# Autodesk Inventor assembly: ASY ДМФ 0100 Барабан
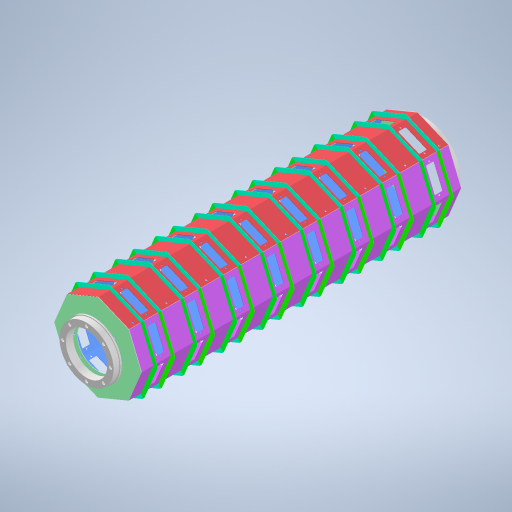
[picture p0: Inventor's stored thumbnail of the model, 512x512]
Saved by Autodesk Inventor 2024.2 (Build 282272000, 272)
## iProperties
Created: 2024-04-28
Part Number: ASY ДМФ 0100 Барабан
Document SubType Name: Assembly
Designer: pokla
Author: pokla
## Documents named in this file (25)
- C:\Users\admin\Documents\Inventor\DMF-Disk-Micro-Filter\ASY ДМФ 0100 Барабан.iam
- C:\Users\admin\Documents\Inventor\DMF-Disk-Micro-Filter\ДМФ 01 21 Барабан торец НОС.ipt
- C:\Users\admin\Documents\Inventor\DMF-Disk-Micro-Filter\ДМФ 01 13 Барабан Лист лев брт.ipt
- C:\Users\admin\Documents\Inventor\DMF-Disk-Micro-Filter\ДМФ 01 14 Барабан Лист прав брт.ipt
- C:\Users\admin\Documents\Inventor\DMF-Disk-Micro-Filter\ДМФ 01 31 Барабан Опорное кольцо НОС.ipt
- C:\Users\admin\Documents\Inventor\DMF-Disk-Micro-Filter\ДМФ 01 17 опора крышки.ipt
- C:\Users\admin\Documents\Inventor\DMF-Disk-Micro-Filter\ДМС 000 размеры.ipt
- C:\Users\admin\Documents\Inventor\DMF-Disk-Micro-Filter\ДМФ 01 41 Шестерня ведомая.ipt
- C:\Users\admin\Documents\Inventor\DMF-Disk-Micro-Filter\ДМФ 01 12 Барабан усилитель.ipt
- C:\Users\admin\Documents\Inventor\DMF-Disk-Micro-Filter\ASY ДМФ 010 крышка.iam
- C:\Users\admin\Documents\Inventor\DMF-Disk-Micro-Filter\ДМФ 01 32 Барабан Опорное кольцо КОРМА.ipt
- C:\Users\admin\Documents\Inventor\DMF-Disk-Micro-Filter\ДМФ 01 22 Барабан торец КОРМА.ipt
- C:\Users\admin\Documents\Inventor\DMF-Disk-Micro-Filter\ASY ДМФ 01 50 Кассета.iam
- ДМС 103 Опорное кольцо вала хвост.ipt
- C:\Users\admin\Documents\Inventor\DMF-Disk-Micro-Filter\ДМС 101 Барабан торец.ipt
- C:\Users\admin\Documents\Inventor\DMF-Disk-Micro-Filter\ДМФ 011 Барабан Лист левый борт.ipt
- C:\Users\admin\Documents\Inventor\DMF-Disk-Micro-Filter\ДМФ 012 Барабан Лист прав брт.ipt
- C:\Users\admin\Documents\Inventor\DMF-Disk-Micro-Filter\ДМС 102 Опорное кольцо вала перед.ipt
- C:\Users\admin\Documents\Inventor\DMF-Disk-Micro-Filter\ДМС 103 Полка для крышки.ipt
- C:\Users\admin\Documents\Inventor\DMF-Disk-Micro-Filter\ДМС 105 Шестерня ведомая.ipt
- C:\Users\admin\Documents\Inventor\DMF-Disk-Micro-Filter\ДМФ 0112 Сектор кольца усилителя барабана_CPY.ipt
- C:\Users\admin\Documents\Inventor\DMF-Disk-Micro-Filter\ASY ДМФ 0110 крышка галка.iam
- C:\Users\admin\Documents\Inventor\DMF-Disk-Micro-Filter\ДМС 103 Опорное кольцо вала хвост.ipt.ipt
- C:\Users\admin\Documents\Inventor\DMF-Disk-Micro-Filter\ДМС 101 Барабан торец зад.ipt
- C:\Users\admin\Documents\Inventor\DMF-Disk-Micro-Filter\ASY ДМФ 0120 Кассета.iam
## Components (123 placed, 12 different names)
1. ДМС 000 размеры:1
2. ДМС 102 Опорное кольцо вала перед:1 — Mate:1, Mate:2, Rotational:4, Mate:6, Rotational:5
3. ДМС 103 Опорное кольцо вала хвост.ipt:1 — Rotational:7, Mate:14
4. ДМС 101 Барабан торец:2 — Rotational:5, Mate:7, Rigid:15, Rigid:16, Mate:8, Flush:1, Flush:2, Mate:9, Flush:3, Flush:4, Mate:10, Flush:5, Flush:6, Rotational:6
5. ДМФ 011 Барабан Лист левый борт:1 — Rigid:15, Mate:12, Flush:7
6. ДМФ 012 Барабан Лист прав брт:1 — Rigid:16, Mate:11
7. ДМС 103 Полка для крышки:1 — Mate:9, Flush:3, Flush:4
8. ДМС 103 Полка для крышки:2 — Mate:8, Flush:1, Flush:2
9. ДМС 105 Шестерня ведомая:1 — Rotational:4, Mate:6
10. ASY ДМФ 0110 крышка галка:1 [sub-assembly] — Mate:10, Flush:5, Flush:6
11. ДМС 101 Барабан торец зад:1 — Rotational:6, Mate:13, Rotational:7
12. ДМФ 0112 Сектор кольца усилителя барабана_CPY:4 — Rigid:10
13. ДМФ 0112 Сектор кольца усилителя барабана_CPY:1 — Rigid:8
14. ДМФ 0112 Сектор кольца усилителя барабана_CPY:5 — Rigid:10, Rigid:11, Rigid:14
15. ДМФ 0112 Сектор кольца усилителя барабана_CPY:2 — Rigid:8, Rigid:9, Rigid:14
16. ДМФ 0112 Сектор кольца усилителя барабана_CPY:3 — Rigid:9, Mate:12
17. ДМФ 0112 Сектор кольца усилителя барабана_CPY:6 — Rigid:11
18. ДМФ 0112 Сектор кольца усилителя барабана_CPY:7
19. ДМФ 0112 Сектор кольца усилителя барабана_CPY:8
20. ДМФ 0112 Сектор кольца усилителя барабана_CPY:21
21. ДМФ 0112 Сектор кольца усилителя барабана_CPY:28
22. ДМФ 0112 Сектор кольца усилителя барабана_CPY:35
23. ДМФ 0112 Сектор кольца усилителя барабана_CPY:42
24. ДМФ 0112 Сектор кольца усилителя барабана_CPY:9
25. ДМФ 0112 Сектор кольца усилителя барабана_CPY:10
26. ДМФ 0112 Сектор кольца усилителя барабана_CPY:22
27. ДМФ 0112 Сектор кольца усилителя барабана_CPY:29
28. ДМФ 0112 Сектор кольца усилителя барабана_CPY:36
29. ДМФ 0112 Сектор кольца усилителя барабана_CPY:43
30. ДМФ 0112 Сектор кольца усилителя барабана_CPY:11
31. ДМФ 0112 Сектор кольца усилителя барабана_CPY:12
32. ДМФ 0112 Сектор кольца усилителя барабана_CPY:23
33. ДМФ 0112 Сектор кольца усилителя барабана_CPY:30
34. ДМФ 0112 Сектор кольца усилителя барабана_CPY:37
35. ДМФ 0112 Сектор кольца усилителя барабана_CPY:44
36. ДМФ 0112 Сектор кольца усилителя барабана_CPY:13
37. ДМФ 0112 Сектор кольца усилителя барабана_CPY:14
38. ДМФ 0112 Сектор кольца усилителя барабана_CPY:24
39. ДМФ 0112 Сектор кольца усилителя барабана_CPY:31
40. ДМФ 0112 Сектор кольца усилителя барабана_CPY:38
41. ДМФ 0112 Сектор кольца усилителя барабана_CPY:45
42. ДМФ 0112 Сектор кольца усилителя барабана_CPY:15
43. ДМФ 0112 Сектор кольца усилителя барабана_CPY:16
44. ДМФ 0112 Сектор кольца усилителя барабана_CPY:25
45. ДМФ 0112 Сектор кольца усилителя барабана_CPY:32
46. ДМФ 0112 Сектор кольца усилителя барабана_CPY:39
47. ДМФ 0112 Сектор кольца усилителя барабана_CPY:46
48. ДМФ 0112 Сектор кольца усилителя барабана_CPY:17
49. ДМФ 0112 Сектор кольца усилителя барабана_CPY:18
50. ДМФ 0112 Сектор кольца усилителя барабана_CPY:26
51. ДМФ 0112 Сектор кольца усилителя барабана_CPY:33
52. ДМФ 0112 Сектор кольца усилителя барабана_CPY:40
53. ДМФ 0112 Сектор кольца усилителя барабана_CPY:47
54. ДМФ 0112 Сектор кольца усилителя барабана_CPY:19 — Mate:11
55. ДМФ 0112 Сектор кольца усилителя барабана_CPY:20
56. ДМФ 0112 Сектор кольца усилителя барабана_CPY:27
57. ДМФ 0112 Сектор кольца усилителя барабана_CPY:34
58. ДМФ 0112 Сектор кольца усилителя барабана_CPY:41
59. ДМФ 0112 Сектор кольца усилителя барабана_CPY:48 — Flush:7
60. ASY ДМФ 0120 Кассета:1 [sub-assembly]
61. ASY ДМФ 0120 Кассета:2 [sub-assembly]
62. ASY ДМФ 0120 Кассета:3 [sub-assembly]
63. ASY ДМФ 0120 Кассета:4 [sub-assembly]
64. ASY ДМФ 0120 Кассета:5 [sub-assembly]
65. ASY ДМФ 0120 Кассета:6 [sub-assembly]
66. ASY ДМФ 0120 Кассета:7 [sub-assembly]
67. ASY ДМФ 0120 Кассета:8 [sub-assembly]
68. ASY ДМФ 0120 Кассета:9 [sub-assembly]
69. ASY ДМФ 0120 Кассета:10 [sub-assembly]
70. ASY ДМФ 0120 Кассета:11 [sub-assembly]
71. ASY ДМФ 0120 Кассета:12 [sub-assembly]
72. ASY ДМФ 0120 Кассета:13 [sub-assembly]
73. ASY ДМФ 0120 Кассета:14 [sub-assembly]
74. ASY ДМФ 0120 Кассета:15 [sub-assembly]
75. ASY ДМФ 0120 Кассета:16 [sub-assembly]
76. ASY ДМФ 0120 Кассета:17 [sub-assembly]
77. ASY ДМФ 0120 Кассета:18 [sub-assembly]
78. ASY ДМФ 0120 Кассета:19 [sub-assembly]
79. ASY ДМФ 0120 Кассета:20 [sub-assembly]
80. ASY ДМФ 0120 Кассета:21 [sub-assembly]
81. ASY ДМФ 0120 Кассета:22 [sub-assembly]
82. ASY ДМФ 0120 Кассета:23 [sub-assembly]
83. ASY ДМФ 0120 Кассета:24 [sub-assembly]
84. ASY ДМФ 0120 Кассета:25 [sub-assembly]
85. ASY ДМФ 0120 Кассета:26 [sub-assembly]
86. ASY ДМФ 0120 Кассета:27 [sub-assembly]
87. ASY ДМФ 0120 Кассета:28 [sub-assembly]
88. ASY ДМФ 0120 Кассета:29 [sub-assembly]
89. ASY ДМФ 0120 Кассета:30 [sub-assembly]
90. ASY ДМФ 0120 Кассета:31 [sub-assembly]
91. ASY ДМФ 0120 Кассета:32 [sub-assembly]
92. ASY ДМФ 0120 Кассета:33 [sub-assembly]
93. ASY ДМФ 0120 Кассета:34 [sub-assembly]
94. ASY ДМФ 0120 Кассета:35 [sub-assembly]
95. ASY ДМФ 0120 Кассета:36 [sub-assembly]
96. ASY ДМФ 0120 Кассета:37 [sub-assembly]
97. ASY ДМФ 0120 Кассета:38 [sub-assembly]
98. ASY ДМФ 0120 Кассета:39 [sub-assembly]
99. ASY ДМФ 0120 Кассета:40 [sub-assembly]
100. ASY ДМФ 0120 Кассета:41 [sub-assembly]
101. ASY ДМФ 0120 Кассета:42 [sub-assembly]
102. ASY ДМФ 0120 Кассета:43 [sub-assembly]
103. ASY ДМФ 0120 Кассета:44 [sub-assembly]
104. ASY ДМФ 0120 Кассета:45 [sub-assembly]
105. ASY ДМФ 0120 Кассета:46 [sub-assembly]
106. ASY ДМФ 0120 Кассета:47 [sub-assembly]
107. ASY ДМФ 0120 Кассета:48 [sub-assembly]
108. ASY ДМФ 0120 Кассета:49 [sub-assembly]
109. ASY ДМФ 0120 Кассета:50 [sub-assembly]
110. ASY ДМФ 0120 Кассета:51 [sub-assembly]
111. ASY ДМФ 0120 Кассета:52 [sub-assembly]
112. ASY ДМФ 0120 Кассета:53 [sub-assembly]
113. ASY ДМФ 0120 Кассета:54 [sub-assembly]
114. ASY ДМФ 0120 Кассета:55 [sub-assembly]
115. ASY ДМФ 0120 Кассета:56 [sub-assembly]
116. ASY ДМФ 0120 Кассета:57 [sub-assembly]
117. ASY ДМФ 0120 Кассета:58 [sub-assembly]
118. ASY ДМФ 0120 Кассета:59 [sub-assembly]
119. ASY ДМФ 0120 Кассета:60 [sub-assembly]
120. ASY ДМФ 0120 Кассета:61 [sub-assembly]
121. ASY ДМФ 0120 Кассета:62 [sub-assembly]
122. ASY ДМФ 0120 Кассета:63 [sub-assembly]
123. ASY ДМФ 0120 Кассета:64 [sub-assembly]
## Component patterns: (8 elements, first: ДМФ 0112 Сектор кольца усилителя барабана_CPY:4 + ДМФ 0112 Сектор кольца усилителя барабана_CPY:1 + ДМФ 0112 Сектор кольца усилителя барабана_CPY:5 + ДМФ 0112 Сектор кольца усилителя барабана_CPY:2 + ДМФ 0112 Сектор кольца усилителя барабана_CPY:3 + ДМФ 0112 Сектор кольца усилителя барабана_CPY:6), (8 elements), (8 elements, first: ASY ДМФ 0120 Кассета:1), Component Pattern 13:2 (8 elements), Component Pattern 13:3 (8 elements), Component Pattern 13:4 (8 elements), Component Pattern 13:5 (8 elements), Component Pattern 13:6 (8 elements), Component Pattern 13:7 (8 elements), Component Pattern 13:8 (8 elements)
## Relationships (30: Mate 11, WeldJoint 8, Flush 7, RevoluteJoint 4)
- Rigid:8 [WeldJoint]: ДМФ 0112 Сектор кольца усилителя барабана_CPY:1 ↔ ДМФ 0112 Сектор кольца усилителя барабана_CPY:2
- Rigid:9 [WeldJoint]: ДМФ 0112 Сектор кольца усилителя барабана_CPY:2 ↔ ДМФ 0112 Сектор кольца усилителя барабана_CPY:3
- Rigid:10 [WeldJoint]: ДМФ 0112 Сектор кольца усилителя барабана_CPY:4 ↔ ДМФ 0112 Сектор кольца усилителя барабана_CPY:5
- Rigid:11 [WeldJoint]: ДМФ 0112 Сектор кольца усилителя барабана_CPY:5 ↔ ДМФ 0112 Сектор кольца усилителя барабана_CPY:6
- Rigid:14 [WeldJoint] (108 mm): ДМФ 0112 Сектор кольца усилителя барабана_CPY:5 ↔ ДМФ 0112 Сектор кольца усилителя барабана_CPY:2
- Mate:1: ДМС 102 Опорное кольцо вала перед:1
- Mate:2: ДМС 102 Опорное кольцо вала перед:1
- Rotational:4 [RevoluteJoint]: ДМС 102 Опорное кольцо вала перед:1 ↔ ДМС 105 Шестерня ведомая:1
- Mate:6: ДМС 102 Опорное кольцо вала перед:1 ↔ ДМС 105 Шестерня ведомая:1
- Rotational:5 [RevoluteJoint] (24 mm): ДМС 102 Опорное кольцо вала перед:1 ↔ ДМС 101 Барабан торец:2
- Mate:7: ДМС 101 Барабан торец:2
- Rigid:15 [WeldJoint]: ДМС 101 Барабан торец:2 ↔ ДМФ 011 Барабан Лист левый борт:1
- Rigid:16 [WeldJoint]: ДМС 101 Барабан торец:2 ↔ ДМФ 012 Барабан Лист прав брт:1
- Mate:8: ДМС 101 Барабан торец:2 ↔ ДМС 103 Полка для крышки:2
- Flush:1 (2 mm): ДМС 101 Барабан торец:2 ↔ ДМС 103 Полка для крышки:2
- Flush:2 (2 mm): ДМС 101 Барабан торец:2 ↔ ДМС 103 Полка для крышки:2
- Mate:9: ДМС 101 Барабан торец:2 ↔ ДМС 103 Полка для крышки:1
- Flush:3 (2 mm): ДМС 101 Барабан торец:2 ↔ ДМС 103 Полка для крышки:1
- Flush:4 (2 mm): ДМС 101 Барабан торец:2 ↔ ДМС 103 Полка для крышки:1
- Mate:10: ДМС 101 Барабан торец:2 ↔ ASY ДМФ 0110 крышка галка:1
- Flush:5: ДМС 101 Барабан торец:2 ↔ ASY ДМФ 0110 крышка галка:1
- Flush:6: ДМС 101 Барабан торец:2 ↔ ASY ДМФ 0110 крышка галка:1
- Mate:11: ДМФ 012 Барабан Лист прав брт:1 ↔ ДМФ 0112 Сектор кольца усилителя барабана_CPY:19
- Mate:12: ДМФ 011 Барабан Лист левый борт:1 ↔ ДМФ 0112 Сектор кольца усилителя барабана_CPY:3
- Flush:7 (29 mm): ДМФ 011 Барабан Лист левый борт:1 ↔ ДМФ 0112 Сектор кольца усилителя барабана_CPY:48
- [WeldJoint] (5 mm): ASY ДМФ 0110 крышка галка:1 ↔ ASY ДМФ 0120 Кассета:1
- Rotational:6 [RevoluteJoint] (2006 mm): ДМС 101 Барабан торец:2 ↔ ДМС 101 Барабан торец зад:1
- Mate:13: ДМС 101 Барабан торец зад:1
- Rotational:7 [RevoluteJoint]: ДМС 103 Опорное кольцо вала хвост.ipt:1 ↔ ДМС 101 Барабан торец зад:1
- Mate:14: ДМС 103 Опорное кольцо вала хвост.ipt:1
